# Autodesk Inventor assembly: Synchronous Belts Transmission
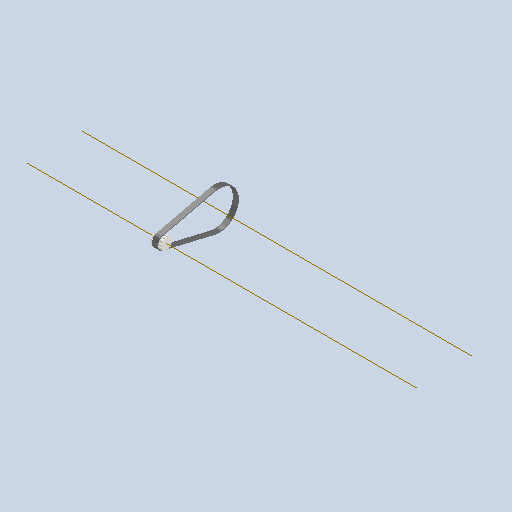
[picture p0: Inventor's stored thumbnail of the model, 512x512]
Saved by Autodesk Inventor 2022.2 (Build 262287000, 287)
## iProperties
ClientObjectVersion: 1
Created: 2022-01-10
Part Number: Synchronous Belts Transmission
Document SubType Name: Assembly
Designer: Jochen
Author: Jochen
## Documents named in this file (3)
- D:\Projects\Lisbeth\CAD\Hip\Hip\Design Accelerator\Synchronous Belts Transmission1.iam
- D:\Projects\Lisbeth\CAD\Hip\Hip\Design Accelerator\Synchronous Belt1.ipt
- D:\Projects\Lisbeth\CAD\Hip\Hip\Design Accelerator\Synchronous Pulley11.ipt
## Components (2 placed, 2 different names)
1. Synchronous Belt:1 — Flush:1, Mate:1, Mate:2
2. Synchronous Pulley1:1 — Flush:1, Mate:1, Mate:2
## Relationships (3: Mate 2, Flush 1)
- Flush:1: Synchronous Belt:1 ↔ Synchronous Pulley1:1
- Mate:1: Synchronous Belt:1 ↔ Synchronous Pulley1:1
- Mate:2: Synchronous Belt:1 ↔ Synchronous Pulley1:1
